# Autodesk Inventor assembly: Cube 1x1 V5 (USB Laser)
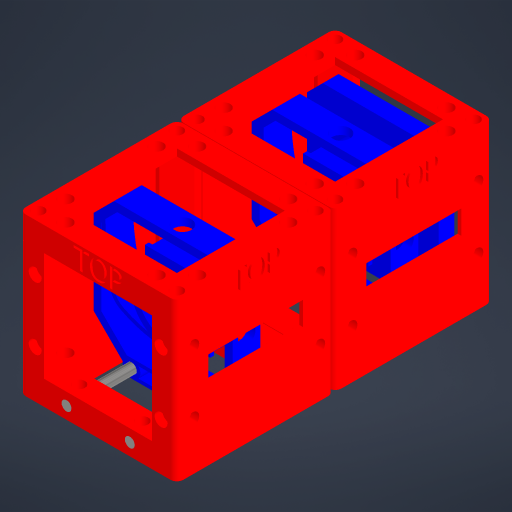
[picture p0: Inventor's stored thumbnail of the model, 512x512]
Saved by Autodesk Inventor 2023.4 (Build 274418000, 418)
## iProperties
Created: 2022-08-13
Part Number: Cube 1x1 V5 (USB Laser)
Document SubType Name: Assembly
Designer: xSibe
Author: xSibe
## Documents named in this file (5)
- C:\.Laptop\.Work\Projects\Project Protocube\Protocube\CAD, STL, OBJ Files\1 CAD\Laser\Cube 1x1 V5 (USB Laser).iam
- C:\.Laptop\.Work\Projects\Project Protocube\Protocube\CAD, STL, OBJ Files\1 CAD\Accessories\Mounting Bar.ipt
- C:\.Laptop\.Work\Projects\Project Protocube\Protocube\CAD, STL, OBJ Files\1 CAD\Filter\Filter Mount (SM1).ipt
- C:\.Laptop\.Work\Projects\Project Protocube\Protocube\CAD, STL, OBJ Files\1 CAD\Laser\Laser Holder (USB Laser).ipt
- C:\.Laptop\.Work\Projects\Project Protocube\Protocube\CAD, STL, OBJ Files\1 CAD\Cubes\Cube 1x1 V5 Laser.iam
## Components (7 placed, 4 different names)
1. Filter Mount (SM1):1 — Mate:4, Mate:5, Mate:8
2. Cube 1x1 V5 Laser:1 [sub-assembly]
3. Laser Holder (USB Laser):1 — Mate:6, Mate:7, Flush:2
4. Mounting Bar:1 — Flush:1, Mate:4, Mate:5, Mate:6, Mate:7
5. Cube 1x1 V5 Laser:2 [sub-assembly] — Mate:8
6. Laser Holder (USB Laser):2
7. Mounting Bar:2
## Component patterns: (2 elements, first: Cube 1x1 V5 Laser:1 + Laser Holder (USB Laser):1 + Mounting Bar:1)
## Relationships (7: Mate 5, Flush 2)
- Flush:1: Mounting Bar:1
- Mate:4: Filter Mount (SM1):1 ↔ Mounting Bar:1
- Mate:5: Filter Mount (SM1):1 ↔ Mounting Bar:1
- Mate:6: Laser Holder (USB Laser):1 ↔ Mounting Bar:1
- Mate:7: Laser Holder (USB Laser):1 ↔ Mounting Bar:1
- Flush:2: Laser Holder (USB Laser):1
- Mate:8: Filter Mount (SM1):1 ↔ Cube 1x1 V5 Laser:2
